# Autodesk Inventor assembly: Assembly-PCB Alone
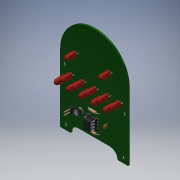
[picture p0: Inventor's stored thumbnail of the model, 180x180]
Saved by Autodesk Inventor 2018 (Build 220112000, 112)
## iProperties
Created: 2019-08-16
Part Number: Assembly-PCB Alone
Document SubType Name: Assembly
Designer: Jamal Bouajjaj
Author: Jamal Bouajjaj
## iProperties of the stored document PinHeader_1x02_P2.54mm_Vertical.iam
Created: 2019-08-16
Part Number: PinHeader_1x02_P2.54mm_Vertical
Document SubType Name: Assembly
Designer: Jamal Bouajjaj
Author: Jamal Bouajjaj
## iProperties of the stored document DIP-8_W7.62mm.ipt
Company: FreeCAD
Created: 2017-03-07
Part Number: DIP-8_W7.62mm
Material: Generic
Description: model of DIP-8_W7.62mm
Document SubType Name: Modeling
Designer: Jamal Bouajjaj
Density: 1 g/cm^3
Appearance: Default
Mass: 0.184953 g
Surface Area: 2.97438 cm^2
Volume: 0.184953 cm^3
Sending System: kicad StepUp
Preprocessor: OCC
Title: DIP-8_W7.62mm.step
Author: kicad StepUp
## iProperties of the stored document DIP-8_W7.62mm_Socket.iam
Created: 2019-08-16
Part Number: DIP-8_W7.62mm_Socket
Document SubType Name: Assembly
Designer: Jamal Bouajjaj
Author: Jamal Bouajjaj
## iProperties of the stored document SOLID_2.ipt
Created: 2019-08-16
Part Number: SOLID_2
Material: Generic
Document SubType Name: Modeling
Designer: Jamal Bouajjaj
Density: 1 g/cm^3
Appearance: Default
Mass: 0.20853 g
Surface Area: 4.37731 cm^2
Volume: 0.20853 cm^3
Author: Jamal Bouajjaj
## iProperties of the stored document LED_D5.0mm.iam
Created: 2019-08-16
Part Number: LED_D5.0mm
Document SubType Name: Assembly
Designer: Jamal Bouajjaj
Author: Jamal Bouajjaj
## iProperties of the stored document SOLID_4.ipt
Created: 2019-08-16
Part Number: SOLID_4
Material: Generic
Document SubType Name: Modeling
Designer: Jamal Bouajjaj
Density: 1 g/cm^3
Appearance: Default
Mass: 0.0393822 g
Surface Area: 1.08508 cm^2
Volume: 0.0393822 cm^3
Author: Jamal Bouajjaj
## iProperties of the stored document SOLID_6.ipt
Created: 2019-08-16
Part Number: SOLID_6
Material: Generic
Document SubType Name: Modeling
Designer: Jamal Bouajjaj
Density: 1 g/cm^3
Appearance: Default
Mass: 0.0180748 g
Surface Area: 0.415451 cm^2
Volume: 0.0180748 cm^3
Author: Jamal Bouajjaj
## iProperties of the stored document COMPOUND.ipt
Created: 2019-08-16
Part Number: COMPOUND
Material: Generic
Document SubType Name: Modeling
Designer: Jamal Bouajjaj
Density: 1 g/cm^3
Appearance: Default
Mass: 9.1095 g
Surface Area: 121.311 cm^2
Volume: 9.1095 cm^3
Author: Jamal Bouajjaj
## iProperties of the stored document SOLID_3.ipt
Created: 2019-08-16
Part Number: SOLID_3
Material: Generic
Document SubType Name: Modeling
Designer: Jamal Bouajjaj
Density: 1 g/cm^3
Appearance: Default
Mass: 0.0300937 g
Surface Area: 0.759695 cm^2
Volume: 0.0300937 cm^3
Author: Jamal Bouajjaj
## iProperties of the stored document SOLID_1.ipt
Created: 2019-08-16
Part Number: SOLID_1
Material: Generic
Document SubType Name: Modeling
Designer: Jamal Bouajjaj
Density: 1 g/cm^3
Appearance: Default
Mass: 0.0300937 g
Surface Area: 0.759695 cm^2
Volume: 0.0300937 cm^3
Author: Jamal Bouajjaj
## iProperties of the stored document CP_Radial_D5.0mm_P2.50mm.iam
Created: 2019-08-16
Part Number: CP_Radial_D5.0mm_P2.50mm
Document SubType Name: Assembly
Designer: Jamal Bouajjaj
Author: Jamal Bouajjaj
## iProperties of the stored document SOLID_5.ipt
Created: 2019-08-16
Part Number: SOLID_5
Material: Generic
Document SubType Name: Modeling
Designer: Jamal Bouajjaj
Density: 1 g/cm^3
Appearance: Default
Mass: 0.155302 g
Surface Area: 1.85065 cm^2
Volume: 0.155302 cm^3
Author: Jamal Bouajjaj
## iProperties of the stored document SOLID.ipt
Created: 2019-10-04
Part Number: SOLID
Material: Generic
Document SubType Name: Modeling
Designer: Electro707
Density: 1 g/cm^3
Appearance: Default
Mass: 0.0929769 g
Surface Area: 1.47718 cm^2
Volume: 0.0929769 cm^3
Author: Electro707
## iProperties of the stored document C_1206_3216Metric.iam
Created: 2019-10-04
Part Number: C_1206_3216Metric
Document SubType Name: Assembly
Designer: Electro707
Author: Electro707
## iProperties of the stored document tht.iam
Created: 2019-10-04
Part Number: tht
Description: KiCad electronic assembly
Document SubType Name: Assembly
Designer: Jamal Bouajjaj
Authority: Unknown
Company: A Company
Sending System: KiCad to STEP converter
Preprocessor: Open CASCADE STEP processor 6.9
Title: tht.step
Author: An Author
## iProperties of the stored document SOLID.ipt
Created: 2019-08-16
Part Number: SOLID
Material: Generic
Document SubType Name: Modeling
Designer: Jamal Bouajjaj
Density: 1 g/cm^3
Appearance: Default
Mass: 0.20853 g
Surface Area: 4.37731 cm^2
Volume: 0.20853 cm^3
Author: Jamal Bouajjaj
## iProperties of the stored document R_Axial_DIN0207_L6.3mm_D2.5mm_P10.16mm_Horizontal.iam
Created: 2019-08-16
Part Number: R_Axial_DIN0207_L6.3mm_D2.5mm_P10.16mm_Horizontal
Document SubType Name: Assembly
Designer: Jamal Bouajjaj
Author: Jamal Bouajjaj
## iProperties of the stored document R_1206_3216Metric.iam
Created: 2019-10-04
Part Number: R_1206_3216Metric
Document SubType Name: Assembly
Designer: Electro707
Author: Electro707
## iProperties of the stored document C_Disc_D3.8mm_W2.6mm_P2.50mm.iam
Created: 2019-08-16
Part Number: C_Disc_D3.8mm_W2.6mm_P2.50mm
Document SubType Name: Assembly
Designer: Jamal Bouajjaj
Author: Jamal Bouajjaj
## Documents named in this file (24)
- **F:\Projects\UNH MakerSpace Kits\2019 - Halloween Event\Ghost\CAD-Inventor\Assembly-PCB Alone.iam*LocalDocs*xDaebae5mFsdbevwzMh25dl2mLc*PinHeader_1x02_P2.54mm_Vertical.iam
- **F:\Projects\UNH MakerSpace Kits\2019 - Halloween Event\Ghost\CAD-Inventor\Assembly-PCB Alone.iam*LocalDocs*xAklsixyoYm2lu04r4mjxxbsyHh*SOLID_4.ipt
- **F:\Projects\UNH MakerSpace Kits\Haloween Board\2019\Ghost\CAD-Inventor\Assembly-PCB Alone.iam*LocalDocs*x3p5cvrpv0gx1epcxXno30iyxUe*DIP-8_W7.62mm.ipt
- **F:\Projects\UNH MakerSpace Kits\2019 - Halloween Event\Ghost\CAD-Inventor\Assembly-PCB Alone.iam*LocalDocs*x2wggqi1oE2bau30qOvx0euv21c*DIP-8_W7.62mm_Socket.iam
- **F:\Projects\UNH MakerSpace Kits\2019 - Halloween Event\Ghost\CAD-Inventor\Assembly-PCB Alone.iam*LocalDocs*x0uagqz1aU4bou30s5215ztdtCa*SOLID_2.ipt
- **F:\Projects\UNH MakerSpace Kits\2019 - Halloween Event\Ghost\CAD-Inventor\Assembly-PCB Alone.iam*LocalDocs*x3el1bvpbMtrduv0zZimo14byEe*LED_D5.0mm.iam
- **F:\Projects\UNH MakerSpace Kits\2019 - Halloween Event\Ghost\CAD-Inventor\Assembly-PCB Alone.iam*LocalDocs*xNzwvlxvzNr13ejktWgyrpvkf3c*SOLID_5.ipt
- **F:\Projects\UNH MakerSpace Kits\2019 - Halloween Event\Ghost\CAD-Inventor\Assembly-PCB Alone.iam*LocalDocs*x41vodokaDjsmu0gpQrgsqcjbTg*SOLID_6.ipt
- **F:\Projects\UNH MakerSpace Kits\2019 - Halloween Event\Ghost\CAD-Inventor\Assembly-PCB Alone.iam*LocalDocs*xAw4kp3jgMsirungcCzbqjs0uSc*COMPOUND.ipt
- **F:\Projects\UNH MakerSpace Kits\2019 - Halloween Event\Ghost\CAD-Inventor\Assembly-PCB Alone.iam*LocalDocs*xP3mrtkn3V4joea0j2brn5gtm5f*SOLID_3.ipt
- **F:\Projects\UNH MakerSpace Kits\2019 - Halloween Event\Ghost\CAD-Inventor\Assembly-PCB Alone.iam*LocalDocs*xKcchf3ug3nqpue4hHt0lxpa2Oc*SOLID_1.ipt
- **F:\Projects\UNH MakerSpace Kits\2019 - Halloween Event\Ghost\CAD-Inventor\Assembly-PCB Alone.iam*LocalDocs*xFj52r5jdWyhqem4r430wnnpr0g*CP_Radial_D5.0mm_P2.50mm.iam
- **F:\Projects\UNH MakerSpace Kits\2019 - Halloween Event\Ghost\CAD-Inventor\Assembly-PCB Alone.iam*LocalDocs*xTetgcy4pO2otelwa3ykfswtzKa*SOLID.ipt
- **F:\Projects\UNH MakerSpace Kits\2019 - Halloween Event\Ghost\CAD-Inventor\Assembly-PCB Alone.iam*LocalDocs*xTbvyi4c45qh3exkbHt2xnfsdOd*C_1206_3216Metric.iam
- **F:\Projects\UNH MakerSpace Kits\2019 - Halloween Event\Ghost\CAD-Inventor\Assembly-PCB Alone.iam*LocalDocs*xUteysuqcGcfvuqosR1jxtsy1Zh*SOLID.ipt
- **F:\Projects\UNH MakerSpace Kits\2019 - Halloween Event\Ghost\CAD-Inventor\Assembly-PCB Alone.iam*LocalDocs*xUwxw5ndr2orlewcuE0a14rjlMh*tht.iam
- **F:\Projects\UNH MakerSpace Kits\2019 - Halloween Event\Ghost\CAD-Inventor\Assembly-PCB Alone.iam*LocalDocs*xXhbfodv5V3lgenoyNxqoupfpLd*R_Axial_DIN0207_L6.3mm_D2.5mm_P10.16mm_Horizontal.iam
- **F:\Projects\UNH MakerSpace Kits\2019 - Halloween Event\Ghost\CAD-Inventor\Assembly-PCB Alone.iam*LocalDocs*xXvjxegcwIxxvu2wrVqzehq0qEc*C_Disc_D3.8mm_W2.6mm_P2.50mm.iam
- **F:\Projects\UNH MakerSpace Kits\2019 - Halloween Event\Ghost\CAD-Inventor\Assembly-PCB Alone.iam*LocalDocs*xX3u3m4bwNsvuedwtJxu21i4lLb*R_1206_3216Metric.iam
- F:\Projects\UNH MakerSpace Kits\2019 - Halloween Event\Ghost\GitHub Folder\CAD-Inventor\Assembly-PCB Alone.iam
- **F:\Projects\UNH MakerSpace Kits\2019 - Halloween Event\Ghost\GitHub Folder\CAD-Inventor\Assembly-PCB Alone.iam*LocalDocs*xUwxw5ndr2orlewcuE0a14rjlMh*tht.iam
- **F:\Projects\UNH MakerSpace Kits\2019 - Halloween Event\Ghost\GitHub Folder\CAD-Inventor\Assembly-PCB Alone.iam*LocalDocs*x3p5cvrpv0gx1epcxXno30iyxUe*DIP-8_W7.62mm.ipt
- F:\Projects\UNH MakerSpace Kits\2019 - Halloween Event\Ghost\GitHub Folder\CAD-Inventor\DIP-8_W7.62mm.step
- F:\Projects\UNH MakerSpace Kits\2019 - Halloween Event\Ghost\GitHub Folder\CAD-Inventor\tht.step
## Components (2 placed, 2 different names)
1. tht:1 [sub-assembly] — Mate:13, Mate:14, Mate:15
2. DIP-8_W7.62mm:1 — Mate:1, Mate:2, Mate:3, Mate:4, Mate:5, Mate:6, Mate:9, Mate:10, Mate:15
## Relationships (15: Mate 15)
- Mate:1: DIP-8_W7.62mm:1
- Mate:2: DIP-8_W7.62mm:1
- Mate:3: DIP-8_W7.62mm:1
- Mate:4: DIP-8_W7.62mm:1
- Mate:5: DIP-8_W7.62mm:1
- Mate:6: DIP-8_W7.62mm:1
- Mate:7
- Mate:8
- Mate:9: DIP-8_W7.62mm:1
- Mate:10: DIP-8_W7.62mm:1
- Mate:11
- Mate:12
- Mate:13: tht:1
- Mate:14: tht:1
- Mate:15: tht:1 ↔ DIP-8_W7.62mm:1
